# Autodesk Inventor assembly: Printhead Assembly REVII
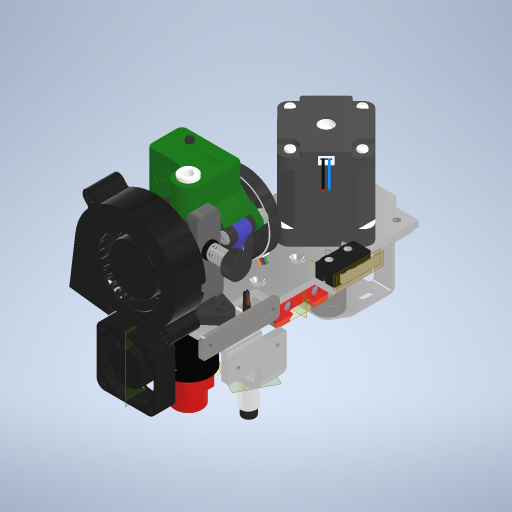
[picture p0: Inventor's stored thumbnail of the model, 512x512]
Saved by Autodesk Inventor 2024 (Build 280153000, 153)
## iProperties
Created: 2023-06-15
Part Number: Printhead Assembly REVII
Document SubType Name: Assembly
Designer: Ishaan
Author: Ishaan
## Documents named in this file (17)
- E:\Projects\Axiom--IDEX-3D-Printer\CAD\01 - Printhead\Printhead Assembly REVII.iam
- E:\Projects\Axiom--IDEX-3D-Printer\CAD\00 - COTS Components\Orbiter Extruder\Orbiter Extruder with Sensor.iam
- E:\Projects\Axiom--IDEX-3D-Printer\CAD\00 - COTS Components\CHC Hotend\TD6S-CHC_mockup.iam
- E:\Projects\Axiom--IDEX-3D-Printer\CAD\00 - COTS Components\3010 Fan\Fan 3010.ipt
- E:\Projects\Axiom--IDEX-3D-Printer\CAD\00 - COTS Components\5015 Fan\Radial-Cooling-Fan-5015-DC12V.iam
- E:\Projects\Axiom--IDEX-3D-Printer\CAD\00 - COTS Components\MGN12H\MGN12H, LINEAR GUIDE BLOCK.ipt
- E:\Projects\Axiom--IDEX-3D-Printer\CAD\00 - COTS Components\Hardware\624 Bearing.ipt
- E:\Projects\Axiom--IDEX-3D-Printer\CAD\00 - COTS Components\Hardware\1127-8-AL.ipt
- E:\Projects\Axiom--IDEX-3D-Printer\CAD\00 - COTS Components\6mm 20T GT2 Timing Pulley 5mm Bore\6mm 20T GT2 Timing Pulley 5mm Bore.ipt
- E:\Projects\Axiom--IDEX-3D-Printer\CAD\00 - COTS Components\Microswitch\MS085xx02FxxxS1A.ipt
- E:\Projects\Axiom--IDEX-3D-Printer\CAD\00 - COTS Components\PINDA Probe\PINDA_placeholder.ipt
- E:\Projects\Axiom--IDEX-3D-Printer\CAD\01 - Printhead\Idler Shear Brace.ipt
- E:\Projects\Axiom--IDEX-3D-Printer\CAD\00 - COTS Components\Hardware\M4 Shim.ipt
- E:\Projects\Axiom--IDEX-3D-Printer\CAD\01 - Printhead\Front Cowling.ipt
- E:\Projects\Axiom--IDEX-3D-Printer\CAD\01 - Printhead\Printhead Base Plate REVII.ipt
- E:\Projects\Axiom--IDEX-3D-Printer\CAD\00 - COTS Components\NEMA 14 - X-Axis Short\14HS17-0504S.ipt
- E:\Projects\Axiom--IDEX-3D-Printer\CAD\01 - Printhead\Cowling Magnetic Catch.ipt
## Components (22 placed, 16 different names)
1. Printhead Base Plate REVII:1 — Insert:27, Insert:28, Insert:29, Insert:30, Insert:31, Insert:32, Insert:33, Insert:34, Insert:37, Insert:38, Insert:41, Insert:42, Insert:43, Insert:44, Mate:13, Mate:14, Flush:6, Angle:1, Insert:49, Insert:50, Insert:51, Insert:52
2. Orbiter Extruder with Sensor:1 [sub-assembly] — Insert:41, Insert:42
3. TD6S-CHC_mockup:1 [sub-assembly] — Flush:2, Insert:43, Insert:44, Mate:15
4. Fan 3010:1 — Insert:45, Insert:46
5. Radial-Cooling-Fan-5015-DC12V:1 [sub-assembly] — Insert:47, Insert:48
6. MGN12H, LINEAR GUIDE BLOCK:1 — Insert:27, Insert:28
7. 624 Bearing:1 — Insert:13, Insert:23
8. 624 Bearing:2 — Insert:13, Insert:17
9. 624 Bearing:3 — Insert:11, Insert:24
10. 624 Bearing:4 — Insert:11, Insert:16
11. 1127-8-AL:1 — Insert:17, Insert:29
12. 1127-8-AL:2 — Insert:16, Insert:30
13. 6mm 20T GT2 Timing Pulley 5mm Bore:1 — Mate:14, Mate:16
14. MS085xx02FxxxS1A:1 — Insert:31, Insert:32
15. MS085xx02FxxxS1A:2 — Insert:33, Insert:34
16. PINDA_placeholder:1 — Flush:2, Flush:5, Mate:13
17. Idler Shear Brace:1 — Insert:25, Insert:26, Insert:37, Insert:38
18. M4 Shim:1 — Insert:24, Insert:25
19. M4 Shim:2 — Insert:23, Insert:26
20. 14HS17-0504S:1 — Insert:49, Insert:50, Mate:16, Insert:51, Insert:52
21. Front Cowling:1 — Mate:15, Flush:6, Angle:1, Insert:45, Insert:46, Insert:47, Insert:48
22. Cowling Magnetic Catch:1
## Relationships (38: Insert 30, Mate 4, Flush 3, Angle 1)
- Insert:11: 624 Bearing:3 ↔ 624 Bearing:4
- Insert:13: 624 Bearing:1 ↔ 624 Bearing:2
- Insert:16: 624 Bearing:4 ↔ 1127-8-AL:2
- Insert:17: 624 Bearing:2 ↔ 1127-8-AL:1
- Flush:2 (-1 mm): TD6S-CHC_mockup:1 ↔ PINDA_placeholder:1
- Insert:23: 624 Bearing:1 ↔ M4 Shim:2
- Insert:24: 624 Bearing:3 ↔ M4 Shim:1
- Insert:25: Idler Shear Brace:1 ↔ M4 Shim:1
- Insert:26: Idler Shear Brace:1 ↔ M4 Shim:2
- Insert:27: Printhead Base Plate REVII:1 ↔ MGN12H, LINEAR GUIDE BLOCK:1
- Insert:28: Printhead Base Plate REVII:1 ↔ MGN12H, LINEAR GUIDE BLOCK:1
- Insert:29: Printhead Base Plate REVII:1 ↔ 1127-8-AL:1
- Insert:30: Printhead Base Plate REVII:1 ↔ 1127-8-AL:2
- Insert:31: Printhead Base Plate REVII:1 ↔ MS085xx02FxxxS1A:1
- Insert:32: Printhead Base Plate REVII:1 ↔ MS085xx02FxxxS1A:1
- Insert:33: Printhead Base Plate REVII:1 ↔ MS085xx02FxxxS1A:2
- Insert:34: Printhead Base Plate REVII:1 ↔ MS085xx02FxxxS1A:2
- Insert:37: Printhead Base Plate REVII:1 ↔ Idler Shear Brace:1
- Insert:38: Printhead Base Plate REVII:1 ↔ Idler Shear Brace:1
- Insert:41: Printhead Base Plate REVII:1 ↔ Orbiter Extruder with Sensor:1
- Insert:42: Printhead Base Plate REVII:1 ↔ Orbiter Extruder with Sensor:1
- Insert:43: Printhead Base Plate REVII:1 ↔ TD6S-CHC_mockup:1
- Insert:44: Printhead Base Plate REVII:1 ↔ TD6S-CHC_mockup:1
- Flush:5 (-18 mm): PINDA_placeholder:1
- Mate:13: Printhead Base Plate REVII:1 ↔ PINDA_placeholder:1
- Mate:14: Printhead Base Plate REVII:1 ↔ 6mm 20T GT2 Timing Pulley 5mm Bore:1
- Mate:15: TD6S-CHC_mockup:1 ↔ Front Cowling:1
- Flush:6: Printhead Base Plate REVII:1 ↔ Front Cowling:1
- Angle:1 (0 deg): Printhead Base Plate REVII:1 ↔ Front Cowling:1
- Insert:45: Fan 3010:1 ↔ Front Cowling:1
- Insert:46: Fan 3010:1 ↔ Front Cowling:1
- Insert:47: Radial-Cooling-Fan-5015-DC12V:1 ↔ Front Cowling:1
- Insert:48: Radial-Cooling-Fan-5015-DC12V:1 ↔ Front Cowling:1
- Insert:49: Printhead Base Plate REVII:1 ↔ 14HS17-0504S:1
- Insert:50: Printhead Base Plate REVII:1 ↔ 14HS17-0504S:1
- Mate:16: 6mm 20T GT2 Timing Pulley 5mm Bore:1 ↔ 14HS17-0504S:1
- Insert:51: Printhead Base Plate REVII:1 ↔ 14HS17-0504S:1
- Insert:52: Printhead Base Plate REVII:1 ↔ 14HS17-0504S:1
